# Autodesk Inventor assembly: LEG2
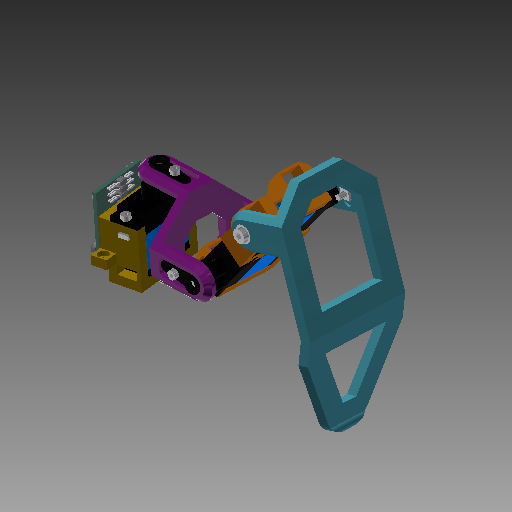
[picture p0: Inventor's stored thumbnail of the model, 512x512]
Saved by Autodesk Inventor 2017 (Build 210142000, 142)
## iProperties
Created: 2018-01-10
Part Number: LEG2
Document SubType Name: Assembly
Designer: Alex
Author: Alex
## Documents named in this file (12)
- C:\Users\Alexander Miller\Documents\Git\HeRo-Mini\Hardware\Assembly\LEG2.iam
- C:\Users\Alexander Miller\Documents\Git\HeRo-Mini\Hardware\Part\Design\FEMUR.ipt
- C:\Users\Alexander Miller\Documents\Git\HeRo-Mini\Hardware\Part\Design\COXA.ipt
- C:\Users\Alexander Miller\Documents\Git\HeRo-Mini\Hardware\Assembly\SERVO.iam
- C:\Users\Alexander Miller\Documents\Git\HeRo-Mini\Hardware\Part\Design\TIBIA.ipt
- C:\Users\Alexander Miller\Documents\Git\HeRo-Mini\Hardware\Part\Hardware\M2_SCREW_8MM.ipt
- C:\Users\Alexander Miller\Documents\Git\HeRo-Mini\Hardware\Part\Hardware\BEARING.ipt
- C:\Users\Alexander Miller\Documents\Git\HeRo-Mini\Hardware\Part\Hardware\M3_SCREW_8MM.ipt
- C:\Users\Alexander Miller\Documents\Git\HeRo-Mini\Hardware\Part\Hardware\NUT_3MM.ipt
- C:\Users\Alexander Miller\Documents\Git\HeRo-Mini\Hardware\Part\Design\HIP.ipt
- C:\Users\Alexander Miller\Documents\Git\HeRo-Mini\Hardware\Assembly\Controller.iam
- C:\Users\Alexander Miller\Documents\Git\HeRo-Mini\Hardware\Part\Hardware\NUT_2MM.ipt
## Components (31 placed, 11 different names)
1. FEMUR:1 — Rigid:1, Rigid:2, Rigid:11, Rigid:13
2. COXA:1 — Rigid:3, Rigid:9, Rigid:18, Rigid:21
3. SERVO:1 [sub-assembly] — Rigid:1, Rigid:3, Rigid:5, Rigid:6, Rigid:28
4. SERVO:2 [sub-assembly] — Rigid:2, Rigid:7, Rigid:8, Rigid:15, Rigid:29
5. TIBIA:1 — Rigid:15, Rigid:16
6. M2_SCREW_8MM:1 — Rigid:8
7. M2_SCREW_8MM:2 — Rigid:7
8. M2_SCREW_8MM:3 — Rigid:6
9. M2_SCREW_8MM:4 — Rigid:5
10. BEARING:1 — Rigid:9
11. BEARING:2 — Rigid:16
12. M3_SCREW_8MM:1 — Rigid:12
13. M3_SCREW_8MM:2 — Rigid:14
14. NUT_3MM:1 — Rigid:13, Rigid:14
15. NUT_3MM:2 — Rigid:11, Rigid:12
16. HIP:1 — Rigid:17, Rigid:19, Rigid:20, Rigid:23, Rigid:25
17. SERVO:3 [sub-assembly] — Rigid:17, Rigid:18, Rigid:24, Rigid:26, Rigid:27
18. Controller:1 [sub-assembly] — Rigid:19
19. BEARING:3 — Rigid:21, Rigid:22
20. M3_SCREW_8MM:3 — Rigid:22
21. NUT_3MM:3 — Rigid:20
22. M2_SCREW_8MM:5 — Rigid:24
23. M2_SCREW_8MM:6 — Rigid:26
24. M2_SCREW_8MM:7 — Rigid:29, Rigid:32
25. M2_SCREW_8MM:8 — Rigid:28, Rigid:31
26. M2_SCREW_8MM:9 — Rigid:27, Rigid:30
27. NUT_2MM:1 — Rigid:23
28. NUT_2MM:2 — Rigid:25
29. NUT_2MM:3 — Rigid:30
30. NUT_2MM:4 — Rigid:32
31. NUT_2MM:5 — Rigid:31
## Relationships (30: WeldJoint 30)
- Rigid:1 [WeldJoint]: FEMUR:1 ↔ SERVO:1
- Rigid:2 [WeldJoint]: FEMUR:1 ↔ SERVO:2
- Rigid:3 [WeldJoint]: COXA:1 ↔ SERVO:1
- Rigid:5 [WeldJoint]: SERVO:1 ↔ M2_SCREW_8MM:4
- Rigid:6 [WeldJoint]: SERVO:1 ↔ M2_SCREW_8MM:3
- Rigid:7 [WeldJoint]: SERVO:2 ↔ M2_SCREW_8MM:2
- Rigid:8 [WeldJoint]: SERVO:2 ↔ M2_SCREW_8MM:1
- Rigid:9 [WeldJoint]: COXA:1 ↔ BEARING:1
- Rigid:11 [WeldJoint]: FEMUR:1 ↔ NUT_3MM:2
- Rigid:12 [WeldJoint]: M3_SCREW_8MM:1 ↔ NUT_3MM:2
- Rigid:13 [WeldJoint]: FEMUR:1 ↔ NUT_3MM:1
- Rigid:14 [WeldJoint]: M3_SCREW_8MM:2 ↔ NUT_3MM:1
- Rigid:15 [WeldJoint]: SERVO:2 ↔ TIBIA:1
- Rigid:16 [WeldJoint]: TIBIA:1 ↔ BEARING:2
- Rigid:17 [WeldJoint]: HIP:1 ↔ SERVO:3
- Rigid:18 [WeldJoint]: COXA:1 ↔ SERVO:3
- Rigid:19 [WeldJoint]: HIP:1 ↔ Controller:1
- Rigid:20 [WeldJoint]: HIP:1 ↔ NUT_3MM:3
- Rigid:21 [WeldJoint]: COXA:1 ↔ BEARING:3
- Rigid:22 [WeldJoint]: BEARING:3 ↔ M3_SCREW_8MM:3
- Rigid:23 [WeldJoint]: HIP:1 ↔ NUT_2MM:1
- Rigid:24 [WeldJoint]: SERVO:3 ↔ M2_SCREW_8MM:5
- Rigid:25 [WeldJoint]: HIP:1 ↔ NUT_2MM:2
- Rigid:26 [WeldJoint]: SERVO:3 ↔ M2_SCREW_8MM:6
- Rigid:27 [WeldJoint]: SERVO:3 ↔ M2_SCREW_8MM:9
- Rigid:28 [WeldJoint]: SERVO:1 ↔ M2_SCREW_8MM:8
- Rigid:29 [WeldJoint]: SERVO:2 ↔ M2_SCREW_8MM:7
- Rigid:30 [WeldJoint]: M2_SCREW_8MM:9 ↔ NUT_2MM:3
- Rigid:31 [WeldJoint]: M2_SCREW_8MM:8 ↔ NUT_2MM:5
- Rigid:32 [WeldJoint]: M2_SCREW_8MM:7 ↔ NUT_2MM:4
